# Autodesk Inventor assembly: Base
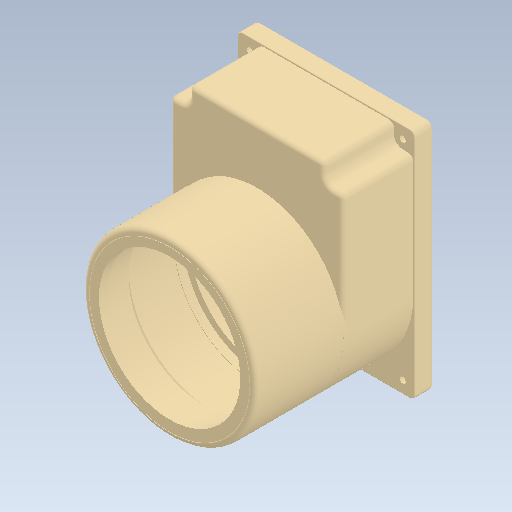
[picture p0: Inventor's stored thumbnail of the model, 512x512]
Saved by Autodesk Inventor 2021 (Build 250183000, 183)
## iProperties
Created: 2020-02-11
Part Number: Base
Document SubType Name: Assembly
Designer: JochenAlt
Author: JochenAlt
## Documents named in this file (3)
- C:\Users\Jochen Alt\Documents\Daten\Projects\MiniBot\CAD\Base.iam
- C:\Users\Jochen Alt\Documents\Daten\Projects\MiniBot\CAD\Base.ipt
- C:\Users\Jochen Alt\Documents\Daten\Projects\MiniBot\CAD\extern\electronics\Odroid C2\ODroid C2.iam
## Components (2 placed, 2 different names)
1. Base:1 — Passend:1, Winkel:1
2. ODroid C2:1 [sub-assembly] — Passend:1, Winkel:1
## Relationships (2: Mate 1, Angle 1)
- Passend:1 [Mate] (5 mm): Base:1 ↔ ODroid C2:1
- Winkel:1 [Angle] (0 deg): Base:1 ↔ ODroid C2:1
